# Autodesk Inventor assembly: Goal Rush W Sensor
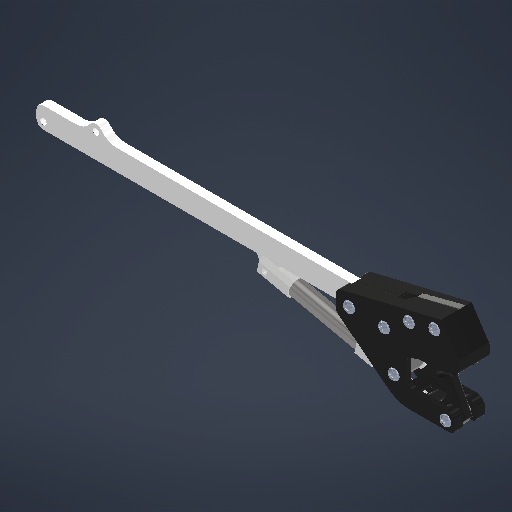
[picture p0: Inventor's stored thumbnail of the model, 512x512]
Saved by Autodesk Inventor 2025 (Build 290162000, 162)
## iProperties
Created: 2025-02-08
Part Number: Goal Rush W Sensor
Document SubType Name: Assembly
Designer: Juan
Author: Juan
## Documents named in this file (18)
- C:\Users\Juan\Documents\GitHub\ATUM-VRC-High-Stakes-CAD\Protobot\Goal Rush W Sensor.iam
- C:\Users\Juan\Documents\GitHub\ATUM-VRC-High-Stakes-CAD\Protobot\Goal Rush U Joint.ipt
- C:\Users\Juan\Documents\GitHub\ATUM-VRC-High-Stakes-CAD\VEX-CAD-Inventor\Motion\Pneumatics\Reference Parts\Pistons\25mm Stroke Pneumatic Cylinder Body.ipt
- C:\Users\Juan\Documents\GitHub\ATUM-VRC-High-Stakes-CAD\VEX-CAD-Inventor\Motion\Pneumatics\Reference Parts\Pistons\25mm Stroke Pneumatic Cylinder Rod.ipt
- C:\Users\Juan\Documents\GitHub\ATUM-VRC-High-Stakes-CAD\VEX-CAD-Inventor\Structure\Standoff\Standoff .50.ipt
- C:\Users\Juan\Documents\GitHub\ATUM-VRC-High-Stakes-CAD\VEX-CAD-Inventor\Structure\Standoff.ipt
- C:\Users\Juan\Documents\GitHub\ATUM-VRC-High-Stakes-CAD\VEX-CAD-Inventor\Motion\Spacers\Washer Teflon\TWasher .375 OD x .06250.ipt
- C:\Users\Juan\Documents\GitHub\ATUM-VRC-High-Stakes-CAD\VEX-CAD-Inventor\Motion\Spacers\Washer Teflon.ipt
- C:\Users\Juan\Documents\GitHub\ATUM-VRC-High-Stakes-CAD\VEX-CAD-Inventor\Structure\Hardware\Screw Steel - Star\SScrew Star Smooth .875.ipt
- C:\Users\Juan\Documents\GitHub\ATUM-VRC-High-Stakes-CAD\VEX-CAD-Inventor\Structure\Hardware\Screw Steel - Star.ipt
- C:\Users\Juan\Documents\GitHub\ATUM-VRC-High-Stakes-CAD\VEX-CAD-Inventor\Structure\Hardware\Nut Thin Nylock.ipt
- C:\Users\Juan\Documents\GitHub\ATUM-VRC-High-Stakes-CAD\VEX-CAD-Inventor\Structure\Hardware\Coupler\Coupler Star .5.ipt
- C:\Users\Juan\Documents\GitHub\ATUM-VRC-High-Stakes-CAD\VEX-CAD-Inventor\Structure\Hardware\Coupler.ipt
- C:\Users\Juan\Documents\GitHub\ATUM-VRC-High-Stakes-CAD\VEX-CAD-Inventor\Electronics\Sensors\Limit Switch.ipt
- C:\Users\Juan\Documents\GitHub\ATUM-VRC-High-Stakes-CAD\Protobot\Goal Jaw Tooth v4.ipt
- C:\Users\Juan\Documents\GitHub\ATUM-VRC-High-Stakes-CAD\Protobot\Goal Jaw Chassis Inner W Sensor.ipt
- C:\Users\Juan\Documents\GitHub\ATUM-VRC-High-Stakes-CAD\Additional Parts\PolyCarb W Sensor.ipt
- C:\Users\Juan\Documents\GitHub\ATUM-VRC-High-Stakes-CAD\Protobot\Goal Jaw Chassis Outer W sensor unlinked.ipt
## Components (23 placed, 13 different names)
1. PolyCarb W Sensor:1 — Mate:6, Flush:3, Mate:28, Mate:29, Mate:30
2. Goal Jaw Tooth v4:1 — Mate:9, Mate:23
3. Goal Rush U Joint:1 — Mate:8, Flush:4, Mate:9, Mate:24
4. 25mm Stroke Pneumatic Cylinder Body:1 — Mate:6, Flush:3, Mate:7
5. 25mm Stroke Pneumatic Cylinder Rod:1 — Mate:7, Mate:8, Flush:4
6. Standoff .50:1 — Mate:12, Mate:13, Mate:14
7. TWasher .375 OD x .06250:1 — Mate:13, Mate:14
8. TWasher .375 OD x .06250:2 — Mate:12
9. Goal Jaw Chassis Outer W sensor unlinked:1 — Mate:23, Rigid:3, Rigid:4, Mate:25, Mate:26, Rigid:5, Rigid:7, Rigid:8, Mate:28, Mate:29, Mate:30, Rigid:9
10. Goal Jaw Chassis Inner W Sensor:1 — Mate:27
11. SScrew Star Smooth .875:2 — Rigid:3
12. SScrew Star Smooth .875:4 — Rigid:4
13. Nut Thin Nylock:1
14. Nut Thin Nylock:2
15. Nut Thin Nylock:3
16. Coupler Star .5:1 — Mate:24
17. Limit Switch:1 — Mate:25, Mate:26, Mate:27, Mate:32, Mate:34
18. SScrew Star Smooth .875:5 — Rigid:9
19. SScrew Star Smooth .875:6 — Rigid:5
20. Nut Thin Nylock:4 — Mate:31, Mate:32
21. Nut Thin Nylock:5 — Mate:33, Mate:34
22. SScrew Star Smooth .875:7 — Rigid:8, Mate:31
23. SScrew Star Smooth .875:8 — Rigid:7, Mate:33
## Relationships (29: Mate 21, WeldJoint 6, Flush 2)
- Mate:6: PolyCarb W Sensor:1 ↔ 25mm Stroke Pneumatic Cylinder Body:1
- Flush:3 (-2.8194 mm): PolyCarb W Sensor:1 ↔ 25mm Stroke Pneumatic Cylinder Body:1
- Mate:7: 25mm Stroke Pneumatic Cylinder Body:1 ↔ 25mm Stroke Pneumatic Cylinder Rod:1
- Mate:8: Goal Rush U Joint:1 ↔ 25mm Stroke Pneumatic Cylinder Rod:1
- Flush:4: Goal Rush U Joint:1 ↔ 25mm Stroke Pneumatic Cylinder Rod:1
- Mate:9: Goal Jaw Tooth v4:1 ↔ Goal Rush U Joint:1
- Mate:12: Standoff .50:1 ↔ TWasher .375 OD x .06250:2
- Mate:13: Standoff .50:1 ↔ TWasher .375 OD x .06250:1
- Mate:14: Standoff .50:1 ↔ TWasher .375 OD x .06250:1
- [Mate]: PolyCarb W Sensor:1 ↔ Goal Jaw Chassis Inner W Sensor:1
- [Mate]: Goal Jaw Tooth v4:1 ↔ Goal Jaw Chassis Inner W Sensor:1
- Mate:23 (0.3969 mm): Goal Jaw Tooth v4:1 ↔ Goal Jaw Chassis Outer W sensor unlinked:1
- Rigid:3 [WeldJoint]: Goal Jaw Chassis Outer W sensor unlinked:1 ↔ SScrew Star Smooth .875:2
- Rigid:4 [WeldJoint]: Goal Jaw Chassis Outer W sensor unlinked:1 ↔ SScrew Star Smooth .875:4
- Mate:24: Goal Rush U Joint:1 ↔ Coupler Star .5:1
- Mate:25: Goal Jaw Chassis Outer W sensor unlinked:1 ↔ Limit Switch:1
- Mate:26: Goal Jaw Chassis Outer W sensor unlinked:1 ↔ Limit Switch:1
- Mate:27: Goal Jaw Chassis Inner W Sensor:1 ↔ Limit Switch:1
- Rigid:5 [WeldJoint]: Goal Jaw Chassis Outer W sensor unlinked:1 ↔ SScrew Star Smooth .875:6
- Rigid:7 [WeldJoint]: Goal Jaw Chassis Outer W sensor unlinked:1 ↔ SScrew Star Smooth .875:8
- Rigid:8 [WeldJoint]: Goal Jaw Chassis Outer W sensor unlinked:1 ↔ SScrew Star Smooth .875:7
- Mate:28: PolyCarb W Sensor:1 ↔ Goal Jaw Chassis Outer W sensor unlinked:1
- Mate:29: PolyCarb W Sensor:1 ↔ Goal Jaw Chassis Outer W sensor unlinked:1
- Mate:30: PolyCarb W Sensor:1 ↔ Goal Jaw Chassis Outer W sensor unlinked:1
- Mate:31: Nut Thin Nylock:4 ↔ SScrew Star Smooth .875:7
- Mate:32: Limit Switch:1 ↔ Nut Thin Nylock:4
- Mate:33: Nut Thin Nylock:5 ↔ SScrew Star Smooth .875:8
- Rigid:9 [WeldJoint]: Goal Jaw Chassis Outer W sensor unlinked:1 ↔ SScrew Star Smooth .875:5
- Mate:34: Limit Switch:1 ↔ Nut Thin Nylock:5
